# Autodesk Inventor assembly: Assembly3
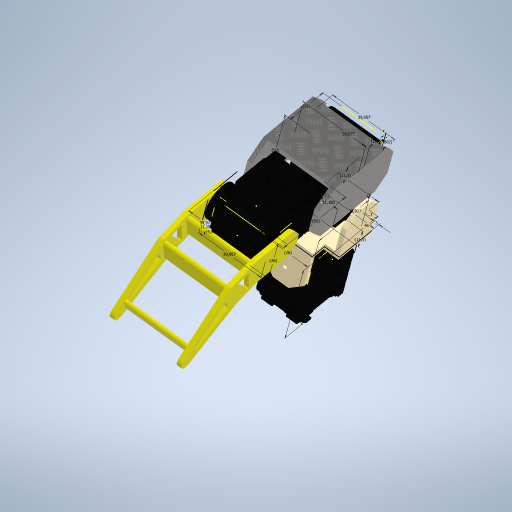
[picture p0: Inventor's stored thumbnail of the model, 512x512]
Saved by Autodesk Inventor 2024 (Build 280153000, 153)
## iProperties
Created: 2024-02-16
Part Number: Assembly3
Document SubType Name: Assembly
Designer: kamil
Author: kamil
## Documents named in this file (5)
- D:\Projects\Robotics\Hexapod\Assembly3.iam
- D:\Projects\Robotics\Hexapod\first_junction.ipt
- D:\Projects\Robotics\Hexapod\AX-12A\AX-12A.iam
- D:\Projects\Robotics\Hexapod\second_junction.ipt
- D:\Projects\Robotics\Hexapod\leg_part.ipt
## Components (6 placed, 4 different names)
1. first_junction:1 — Mate:1, Mate:2, Mate:3, Mate:4, Mate:5, Mate:6, Mate:7
2. AX-12A:1 [sub-assembly] — Mate:1, Mate:2, Mate:3, Mate:4
3. AX-12A:2 [sub-assembly] — Mate:5, Mate:6, Mate:7, Mate:14, Mate:18, Mate:19
4. second_junction:1 — Mate:11, Mate:12, Mate:13, Mate:14, Mate:18, Mate:19
5. AX-12A:3 [sub-assembly] — Mate:11, Mate:12, Mate:13, Mate:15, Mate:16, Mate:17
6. leg_part:1 — Mate:15, Mate:16, Mate:17
## Relationships (16: Mate 16)
- Mate:1: first_junction:1 ↔ AX-12A:1
- Mate:2: first_junction:1 ↔ AX-12A:1
- Mate:3: first_junction:1 ↔ AX-12A:1
- Mate:4: first_junction:1 ↔ AX-12A:1
- Mate:5: first_junction:1 ↔ AX-12A:2
- Mate:6: first_junction:1 ↔ AX-12A:2
- Mate:7: first_junction:1 ↔ AX-12A:2
- Mate:11: second_junction:1 ↔ AX-12A:3
- Mate:12: second_junction:1 ↔ AX-12A:3
- Mate:13: second_junction:1 ↔ AX-12A:3
- Mate:14: AX-12A:2 ↔ second_junction:1
- Mate:15: AX-12A:3 ↔ leg_part:1
- Mate:16: AX-12A:3 ↔ leg_part:1
- Mate:17: AX-12A:3 ↔ leg_part:1
- Mate:18: AX-12A:2 ↔ second_junction:1
- Mate:19: AX-12A:2 ↔ second_junction:1
